# Autodesk Inventor assembly: 566H_plus_Blumotion NL=750 mm Chipboard screws 661.1450.HG 6,3x14,5 L Top row R Top row LD drillings both
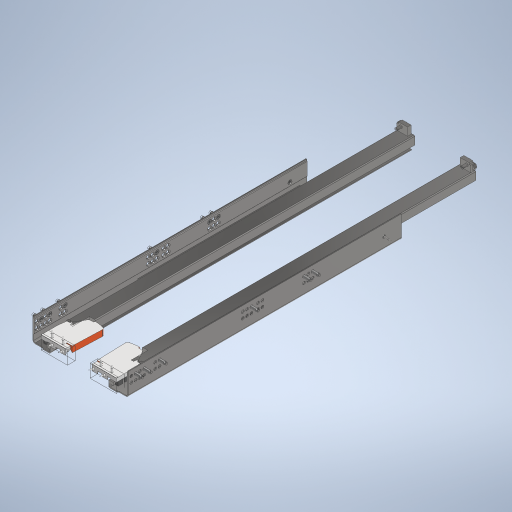
[picture p0: Inventor's stored thumbnail of the model, 512x512]
Saved by Autodesk Inventor 2024 (Build 280153000, 153)
## iProperties
Created: 2019-09-16
Part Number: 566H_plus_Blumotion NL=750 mm Chipboard screws 661.1450.HG 6,3x14,5 L Top row R Top row LD drillings both
Document SubType Name: Assembly
Designer: RokasM
Author: RokasM
## Documents named in this file (296)
- C:\W4INV 2024 Design\LIBRARY\Sliders\Blum TANDEM PLUS BLUMOTION 566 H\566H_iassembly_v1_LD.iam
- C:\W4INV 2024 Design\LIBRARY\Sliders\Blum TANDEM PLUS BLUMOTION 566 H\Blum_TANDEM_PLUS_BLUMOTION_566H.ipt
- C:\W4INV 2024 Design\LIBRARY\Sliders\Blum TANDEM PLUS BLUMOTION 566 H\Lockingdevice.ipt
- C:\W4INV 2024 Design\LIBRARY\Sliders\Blum TANDEM PLUS BLUMOTION 566 H\Locking_device\Locking device L.ipt
- C:\W4INV 2024 Design\LIBRARY\Sliders\Blum TANDEM PLUS BLUMOTION 566 H\Locking_device\Locking device R.ipt
- C:\W4INV 2024 Design\LIBRARY\Sliders\Blum TANDEM PLUS BLUMOTION 566 H\566H\566H7500B01 Chipboard screws top_row L.ipt
- C:\W4INV 2024 Design\LIBRARY\Sliders\Blum TANDEM PLUS BLUMOTION 566 H\566H\566H7500B01 Chipboard screws top_row R.ipt
- C:\W4INV 2020 Design\LIBRARY\Rollers\Blum TANDEM PLUS BLUMOTION 566 H\Lockingdevice.ipt
- 566H_plus_Blumotion NL=450 mm Chipboard screws 4x15 mm L Bottom row R Bottom row LD drillings both.iam
- 566H_plus_Blumotion NL=450 mm Chipboard screws 4x15 mm L Bottom row R Bottom row LD drillings bottom.iam
- 566H_plus_Blumotion NL=450 mm Chipboard screws 4x15 mm L Bottom row R Bottom row LD drillings facade.iam
- 566H_plus_Blumotion NL=450 mm Chipboard screws 4x15 mm L Bottom row R Bottom row LD drillings none.iam
- 566H_plus_Blumotion NL=450 mm Chipboard screws 4x15 mm L Bottom row R Top row LD drillings both.iam
- 566H_plus_Blumotion NL=450 mm Chipboard screws 4x15 mm L Bottom row R Top row LD drillings bottom.iam
- 566H_plus_Blumotion NL=450 mm Chipboard screws 4x15 mm L Bottom row R Top row LD drillings facade.iam
- 566H_plus_Blumotion NL=450 mm Chipboard screws 4x15 mm L Bottom row R Top row LD drillings none.iam
- 566H_plus_Blumotion NL=450 mm Chipboard screws 4x15 mm L Top row R Bottom row LD drillings both.iam
- 566H_plus_Blumotion NL=450 mm Chipboard screws 4x15 mm L Top row R Bottom row LD drillings bottom.iam
- 566H_plus_Blumotion NL=450 mm Chipboard screws 4x15 mm L Top row R Bottom row LD drillings facade.iam
- 566H_plus_Blumotion NL=450 mm Chipboard screws 4x15 mm L Top row R Bottom row LD drillings none.iam
- 566H_plus_Blumotion NL=450 mm Chipboard screws 4x15 mm L Top row R Top row LD drillings both.iam
- 566H_plus_Blumotion NL=450 mm Chipboard screws 4x15 mm L Top row R Top row LD drillings bottom.iam
- 566H_plus_Blumotion NL=450 mm Chipboard screws 4x15 mm L Top row R Top row LD drillings facade.iam
- 566H_plus_Blumotion NL=450 mm Chipboard screws 4x15 mm L Top row R Top row LD drillings none.iam
- 566H_plus_Blumotion NL=450 mm Chipboard screws 661.1450.HG 6,3x14,5 L Bottom row R Bottom row LD drillings both.iam
- 566H_plus_Blumotion NL=450 mm Chipboard screws 661.1450.HG 6,3x14,5 L Bottom row R Bottom row LD drillings bottom.iam
- 566H_plus_Blumotion NL=450 mm Chipboard screws 661.1450.HG 6,3x14,5 L Bottom row R Bottom row LD drillings facade.iam
- 566H_plus_Blumotion NL=450 mm Chipboard screws 661.1450.HG 6,3x14,5 L Bottom row R Bottom row LD drillings none.iam
- 566H_plus_Blumotion NL=450 mm Chipboard screws 661.1450.HG 6,3x14,5 L Bottom row R Top row LD drillings both.iam
- 566H_plus_Blumotion NL=450 mm Chipboard screws 661.1450.HG 6,3x14,5 L Bottom row R Top row LD drillings bottom.iam
- 566H_plus_Blumotion NL=450 mm Chipboard screws 661.1450.HG 6,3x14,5 L Bottom row R Top row LD drillings facade.iam
- 566H_plus_Blumotion NL=450 mm Chipboard screws 661.1450.HG 6,3x14,5 L Bottom row R Top row LD drillings none.iam
- 566H_plus_Blumotion NL=450 mm Chipboard screws 661.1450.HG 6,3x14,5 L Top row R Bottom row LD drillings both.iam
- 566H_plus_Blumotion NL=450 mm Chipboard screws 661.1450.HG 6,3x14,5 L Top row R Bottom row LD drillings bottom.iam
- 566H_plus_Blumotion NL=450 mm Chipboard screws 661.1450.HG 6,3x14,5 L Top row R Bottom row LD drillings facade.iam
- 566H_plus_Blumotion NL=450 mm Chipboard screws 661.1450.HG 6,3x14,5 L Top row R Bottom row LD drillings none.iam
- 566H_plus_Blumotion NL=450 mm Chipboard screws 661.1450.HG 6,3x14,5 L Top row R Top row LD drillings both.iam
- 566H_plus_Blumotion NL=450 mm Chipboard screws 661.1450.HG 6,3x14,5 L Top row R Top row LD drillings bottom.iam
- 566H_plus_Blumotion NL=450 mm Chipboard screws 661.1450.HG 6,3x14,5 L Top row R Top row LD drillings facade.iam
- 566H_plus_Blumotion NL=450 mm Chipboard screws 661.1450.HG 6,3x14,5 L Top row R Top row LD drillings none.iam
- 566H_plus_Blumotion NL=500 mm Chipboard screws 4x15 mm L Bottom row R Bottom row LD drillings both.iam
- 566H_plus_Blumotion NL=500 mm Chipboard screws 4x15 mm L Bottom row R Bottom row LD drillings bottom.iam
- 566H_plus_Blumotion NL=500 mm Chipboard screws 4x15 mm L Bottom row R Bottom row LD drillings facade.iam
- 566H_plus_Blumotion NL=500 mm Chipboard screws 4x15 mm L Bottom row R Bottom row LD drillings none.iam
- 566H_plus_Blumotion NL=500 mm Chipboard screws 4x15 mm L Bottom row R Top row LD drillings both.iam
- 566H_plus_Blumotion NL=500 mm Chipboard screws 4x15 mm L Bottom row R Top row LD drillings bottom.iam
- 566H_plus_Blumotion NL=500 mm Chipboard screws 4x15 mm L Bottom row R Top row LD drillings facade.iam
- 566H_plus_Blumotion NL=500 mm Chipboard screws 4x15 mm L Bottom row R Top row LD drillings none.iam
- 566H_plus_Blumotion NL=500 mm Chipboard screws 4x15 mm L Top row R Bottom row LD drillings both.iam
- 566H_plus_Blumotion NL=500 mm Chipboard screws 4x15 mm L Top row R Bottom row LD drillings bottom.iam
- 566H_plus_Blumotion NL=500 mm Chipboard screws 4x15 mm L Top row R Bottom row LD drillings facade.iam
- 566H_plus_Blumotion NL=500 mm Chipboard screws 4x15 mm L Top row R Bottom row LD drillings none.iam
- 566H_plus_Blumotion NL=500 mm Chipboard screws 4x15 mm L Top row R Top row LD drillings both.iam
- 566H_plus_Blumotion NL=500 mm Chipboard screws 4x15 mm L Top row R Top row LD drillings bottom.iam
- 566H_plus_Blumotion NL=500 mm Chipboard screws 4x15 mm L Top row R Top row LD drillings facade.iam
- 566H_plus_Blumotion NL=500 mm Chipboard screws 4x15 mm L Top row R Top row LD drillings none.iam
- 566H_plus_Blumotion NL=500 mm Chipboard screws 661.1450.HG 6,3x14,5 L Bottom row R Bottom row LD drillings both.iam
- 566H_plus_Blumotion NL=500 mm Chipboard screws 661.1450.HG 6,3x14,5 L Bottom row R Bottom row LD drillings bottom.iam
- 566H_plus_Blumotion NL=500 mm Chipboard screws 661.1450.HG 6,3x14,5 L Bottom row R Bottom row LD drillings facade.iam
- 566H_plus_Blumotion NL=500 mm Chipboard screws 661.1450.HG 6,3x14,5 L Bottom row R Bottom row LD drillings none.iam
- 566H_plus_Blumotion NL=500 mm Chipboard screws 661.1450.HG 6,3x14,5 L Bottom row R Top row LD drillings both.iam
- 566H_plus_Blumotion NL=500 mm Chipboard screws 661.1450.HG 6,3x14,5 L Bottom row R Top row LD drillings bottom.iam
- 566H_plus_Blumotion NL=500 mm Chipboard screws 661.1450.HG 6,3x14,5 L Bottom row R Top row LD drillings facade.iam
- 566H_plus_Blumotion NL=500 mm Chipboard screws 661.1450.HG 6,3x14,5 L Bottom row R Top row LD drillings none.iam
- 566H_plus_Blumotion NL=500 mm Chipboard screws 661.1450.HG 6,3x14,5 L Top row R Bottom row LD drillings both.iam
- 566H_plus_Blumotion NL=500 mm Chipboard screws 661.1450.HG 6,3x14,5 L Top row R Bottom row LD drillings bottom.iam
- 566H_plus_Blumotion NL=500 mm Chipboard screws 661.1450.HG 6,3x14,5 L Top row R Bottom row LD drillings facade.iam
- 566H_plus_Blumotion NL=500 mm Chipboard screws 661.1450.HG 6,3x14,5 L Top row R Bottom row LD drillings none.iam
- 566H_plus_Blumotion NL=500 mm Chipboard screws 661.1450.HG 6,3x14,5 L Top row R Top row LD drillings both.iam
- 566H_plus_Blumotion NL=500 mm Chipboard screws 661.1450.HG 6,3x14,5 L Top row R Top row LD drillings bottom.iam
- 566H_plus_Blumotion NL=500 mm Chipboard screws 661.1450.HG 6,3x14,5 L Top row R Top row LD drillings facade.iam
- 566H_plus_Blumotion NL=500 mm Chipboard screws 661.1450.HG 6,3x14,5 L Top row R Top row LD drillings none.iam
- 566H_plus_Blumotion NL=520 mm Chipboard screws 4x15 mm L Bottom row R Bottom row LD drillings both.iam
- 566H_plus_Blumotion NL=520 mm Chipboard screws 4x15 mm L Bottom row R Bottom row LD drillings bottom.iam
- 566H_plus_Blumotion NL=520 mm Chipboard screws 4x15 mm L Bottom row R Bottom row LD drillings facade.iam
- 566H_plus_Blumotion NL=520 mm Chipboard screws 4x15 mm L Bottom row R Bottom row LD drillings none.iam
- 566H_plus_Blumotion NL=520 mm Chipboard screws 4x15 mm L Bottom row R Top row LD drillings both.iam
- 566H_plus_Blumotion NL=520 mm Chipboard screws 4x15 mm L Bottom row R Top row LD drillings bottom.iam
- 566H_plus_Blumotion NL=520 mm Chipboard screws 4x15 mm L Bottom row R Top row LD drillings facade.iam
- 566H_plus_Blumotion NL=520 mm Chipboard screws 4x15 mm L Bottom row R Top row LD drillings none.iam
- 566H_plus_Blumotion NL=520 mm Chipboard screws 4x15 mm L Top row R Bottom row LD drillings both.iam
- 566H_plus_Blumotion NL=520 mm Chipboard screws 4x15 mm L Top row R Bottom row LD drillings bottom.iam
- 566H_plus_Blumotion NL=520 mm Chipboard screws 4x15 mm L Top row R Bottom row LD drillings facade.iam
- 566H_plus_Blumotion NL=520 mm Chipboard screws 4x15 mm L Top row R Bottom row LD drillings none.iam
- 566H_plus_Blumotion NL=520 mm Chipboard screws 4x15 mm L Top row R Top row LD drillings both.iam
- 566H_plus_Blumotion NL=520 mm Chipboard screws 4x15 mm L Top row R Top row LD drillings bottom.iam
- 566H_plus_Blumotion NL=520 mm Chipboard screws 4x15 mm L Top row R Top row LD drillings facade.iam
- 566H_plus_Blumotion NL=520 mm Chipboard screws 4x15 mm L Top row R Top row LD drillings none.iam
- 566H_plus_Blumotion NL=520 mm Chipboard screws 661.1450.HG 6,3x14,5 L Bottom row R Bottom row LD drillings both.iam
- 566H_plus_Blumotion NL=520 mm Chipboard screws 661.1450.HG 6,3x14,5 L Bottom row R Bottom row LD drillings bottom.iam
- 566H_plus_Blumotion NL=520 mm Chipboard screws 661.1450.HG 6,3x14,5 L Bottom row R Bottom row LD drillings facade.iam
- 566H_plus_Blumotion NL=520 mm Chipboard screws 661.1450.HG 6,3x14,5 L Bottom row R Bottom row LD drillings none.iam
- 566H_plus_Blumotion NL=520 mm Chipboard screws 661.1450.HG 6,3x14,5 L Bottom row R Top row LD drillings both.iam
- 566H_plus_Blumotion NL=520 mm Chipboard screws 661.1450.HG 6,3x14,5 L Bottom row R Top row LD drillings bottom.iam
- 566H_plus_Blumotion NL=520 mm Chipboard screws 661.1450.HG 6,3x14,5 L Bottom row R Top row LD drillings facade.iam
- 566H_plus_Blumotion NL=520 mm Chipboard screws 661.1450.HG 6,3x14,5 L Bottom row R Top row LD drillings none.iam
- 566H_plus_Blumotion NL=520 mm Chipboard screws 661.1450.HG 6,3x14,5 L Top row R Bottom row LD drillings both.iam
- 566H_plus_Blumotion NL=520 mm Chipboard screws 661.1450.HG 6,3x14,5 L Top row R Bottom row LD drillings bottom.iam
- 566H_plus_Blumotion NL=520 mm Chipboard screws 661.1450.HG 6,3x14,5 L Top row R Bottom row LD drillings facade.iam
- 566H_plus_Blumotion NL=520 mm Chipboard screws 661.1450.HG 6,3x14,5 L Top row R Bottom row LD drillings none.iam
- 566H_plus_Blumotion NL=520 mm Chipboard screws 661.1450.HG 6,3x14,5 L Top row R Top row LD drillings both.iam
- 566H_plus_Blumotion NL=520 mm Chipboard screws 661.1450.HG 6,3x14,5 L Top row R Top row LD drillings bottom.iam
- 566H_plus_Blumotion NL=520 mm Chipboard screws 661.1450.HG 6,3x14,5 L Top row R Top row LD drillings facade.iam
- 566H_plus_Blumotion NL=520 mm Chipboard screws 661.1450.HG 6,3x14,5 L Top row R Top row LD drillings none.iam
- 566H_plus_Blumotion NL=550 mm Chipboard screws 4x15 mm L Bottom row R Bottom row LD drillings both.iam
- 566H_plus_Blumotion NL=550 mm Chipboard screws 4x15 mm L Bottom row R Bottom row LD drillings bottom.iam
- 566H_plus_Blumotion NL=550 mm Chipboard screws 4x15 mm L Bottom row R Bottom row LD drillings facade.iam
- 566H_plus_Blumotion NL=550 mm Chipboard screws 4x15 mm L Bottom row R Bottom row LD drillings none.iam
- 566H_plus_Blumotion NL=550 mm Chipboard screws 4x15 mm L Bottom row R Top row LD drillings both.iam
- 566H_plus_Blumotion NL=550 mm Chipboard screws 4x15 mm L Bottom row R Top row LD drillings bottom.iam
- 566H_plus_Blumotion NL=550 mm Chipboard screws 4x15 mm L Bottom row R Top row LD drillings facade.iam
- 566H_plus_Blumotion NL=550 mm Chipboard screws 4x15 mm L Bottom row R Top row LD drillings none.iam
- 566H_plus_Blumotion NL=550 mm Chipboard screws 4x15 mm L Top row R Bottom row LD drillings both.iam
- 566H_plus_Blumotion NL=550 mm Chipboard screws 4x15 mm L Top row R Bottom row LD drillings bottom.iam
- 566H_plus_Blumotion NL=550 mm Chipboard screws 4x15 mm L Top row R Bottom row LD drillings facade.iam
- 566H_plus_Blumotion NL=550 mm Chipboard screws 4x15 mm L Top row R Bottom row LD drillings none.iam
- 566H_plus_Blumotion NL=550 mm Chipboard screws 4x15 mm L Top row R Top row LD drillings both.iam
- 566H_plus_Blumotion NL=550 mm Chipboard screws 4x15 mm L Top row R Top row LD drillings bottom.iam
- 566H_plus_Blumotion NL=550 mm Chipboard screws 4x15 mm L Top row R Top row LD drillings facade.iam
- 566H_plus_Blumotion NL=550 mm Chipboard screws 4x15 mm L Top row R Top row LD drillings none.iam
- 566H_plus_Blumotion NL=550 mm Chipboard screws 661.1450.HG 6,3x14,5 L Bottom row R Bottom row LD drillings both.iam
- 566H_plus_Blumotion NL=550 mm Chipboard screws 661.1450.HG 6,3x14,5 L Bottom row R Bottom row LD drillings bottom.iam
- 566H_plus_Blumotion NL=550 mm Chipboard screws 661.1450.HG 6,3x14,5 L Bottom row R Bottom row LD drillings facade.iam
- 566H_plus_Blumotion NL=550 mm Chipboard screws 661.1450.HG 6,3x14,5 L Bottom row R Bottom row LD drillings none.iam
- 566H_plus_Blumotion NL=550 mm Chipboard screws 661.1450.HG 6,3x14,5 L Bottom row R Top row LD drillings both.iam
- 566H_plus_Blumotion NL=550 mm Chipboard screws 661.1450.HG 6,3x14,5 L Bottom row R Top row LD drillings bottom.iam
- 566H_plus_Blumotion NL=550 mm Chipboard screws 661.1450.HG 6,3x14,5 L Bottom row R Top row LD drillings facade.iam
- 566H_plus_Blumotion NL=550 mm Chipboard screws 661.1450.HG 6,3x14,5 L Bottom row R Top row LD drillings none.iam
- 566H_plus_Blumotion NL=550 mm Chipboard screws 661.1450.HG 6,3x14,5 L Top row R Bottom row LD drillings both.iam
- 566H_plus_Blumotion NL=550 mm Chipboard screws 661.1450.HG 6,3x14,5 L Top row R Bottom row LD drillings bottom.iam
- 566H_plus_Blumotion NL=550 mm Chipboard screws 661.1450.HG 6,3x14,5 L Top row R Bottom row LD drillings facade.iam
- 566H_plus_Blumotion NL=550 mm Chipboard screws 661.1450.HG 6,3x14,5 L Top row R Bottom row LD drillings none.iam
- 566H_plus_Blumotion NL=550 mm Chipboard screws 661.1450.HG 6,3x14,5 L Top row R Top row LD drillings both.iam
- 566H_plus_Blumotion NL=550 mm Chipboard screws 661.1450.HG 6,3x14,5 L Top row R Top row LD drillings bottom.iam
- 566H_plus_Blumotion NL=550 mm Chipboard screws 661.1450.HG 6,3x14,5 L Top row R Top row LD drillings facade.iam
- 566H_plus_Blumotion NL=550 mm Chipboard screws 661.1450.HG 6,3x14,5 L Top row R Top row LD drillings none.iam
- 566H_plus_Blumotion NL=580 mm Chipboard screws 4x15 mm L Bottom row R Bottom row LD drillings both.iam
- 566H_plus_Blumotion NL=580 mm Chipboard screws 4x15 mm L Bottom row R Bottom row LD drillings bottom.iam
- 566H_plus_Blumotion NL=580 mm Chipboard screws 4x15 mm L Bottom row R Bottom row LD drillings facade.iam
- 566H_plus_Blumotion NL=580 mm Chipboard screws 4x15 mm L Bottom row R Bottom row LD drillings none.iam
- 566H_plus_Blumotion NL=580 mm Chipboard screws 4x15 mm L Bottom row R Top row LD drillings both.iam
- 566H_plus_Blumotion NL=580 mm Chipboard screws 4x15 mm L Bottom row R Top row LD drillings bottom.iam
- 566H_plus_Blumotion NL=580 mm Chipboard screws 4x15 mm L Bottom row R Top row LD drillings facade.iam
- 566H_plus_Blumotion NL=580 mm Chipboard screws 4x15 mm L Bottom row R Top row LD drillings none.iam
- 566H_plus_Blumotion NL=580 mm Chipboard screws 4x15 mm L Top row R Bottom row LD drillings both.iam
- 566H_plus_Blumotion NL=580 mm Chipboard screws 4x15 mm L Top row R Bottom row LD drillings bottom.iam
- 566H_plus_Blumotion NL=580 mm Chipboard screws 4x15 mm L Top row R Bottom row LD drillings facade.iam
- 566H_plus_Blumotion NL=580 mm Chipboard screws 4x15 mm L Top row R Bottom row LD drillings none.iam
- 566H_plus_Blumotion NL=580 mm Chipboard screws 4x15 mm L Top row R Top row LD drillings both.iam
- 566H_plus_Blumotion NL=580 mm Chipboard screws 4x15 mm L Top row R Top row LD drillings bottom.iam
- 566H_plus_Blumotion NL=580 mm Chipboard screws 4x15 mm L Top row R Top row LD drillings facade.iam
- 566H_plus_Blumotion NL=580 mm Chipboard screws 4x15 mm L Top row R Top row LD drillings none.iam
- 566H_plus_Blumotion NL=580 mm Chipboard screws 661.1450.HG 6,3x14,5 L Bottom row R Bottom row LD drillings both.iam
- 566H_plus_Blumotion NL=580 mm Chipboard screws 661.1450.HG 6,3x14,5 L Bottom row R Bottom row LD drillings bottom.iam
- 566H_plus_Blumotion NL=580 mm Chipboard screws 661.1450.HG 6,3x14,5 L Bottom row R Bottom row LD drillings facade.iam
- 566H_plus_Blumotion NL=580 mm Chipboard screws 661.1450.HG 6,3x14,5 L Bottom row R Bottom row LD drillings none.iam
- 566H_plus_Blumotion NL=580 mm Chipboard screws 661.1450.HG 6,3x14,5 L Bottom row R Top row LD drillings both.iam
- 566H_plus_Blumotion NL=580 mm Chipboard screws 661.1450.HG 6,3x14,5 L Bottom row R Top row LD drillings bottom.iam
- 566H_plus_Blumotion NL=580 mm Chipboard screws 661.1450.HG 6,3x14,5 L Bottom row R Top row LD drillings facade.iam
- 566H_plus_Blumotion NL=580 mm Chipboard screws 661.1450.HG 6,3x14,5 L Bottom row R Top row LD drillings none.iam
- 566H_plus_Blumotion NL=580 mm Chipboard screws 661.1450.HG 6,3x14,5 L Top row R Bottom row LD drillings both.iam
- 566H_plus_Blumotion NL=580 mm Chipboard screws 661.1450.HG 6,3x14,5 L Top row R Bottom row LD drillings bottom.iam
- 566H_plus_Blumotion NL=580 mm Chipboard screws 661.1450.HG 6,3x14,5 L Top row R Bottom row LD drillings facade.iam
- 566H_plus_Blumotion NL=580 mm Chipboard screws 661.1450.HG 6,3x14,5 L Top row R Bottom row LD drillings none.iam
- 566H_plus_Blumotion NL=580 mm Chipboard screws 661.1450.HG 6,3x14,5 L Top row R Top row LD drillings both.iam
- 566H_plus_Blumotion NL=580 mm Chipboard screws 661.1450.HG 6,3x14,5 L Top row R Top row LD drillings bottom.iam
- 566H_plus_Blumotion NL=580 mm Chipboard screws 661.1450.HG 6,3x14,5 L Top row R Top row LD drillings facade.iam
- 566H_plus_Blumotion NL=580 mm Chipboard screws 661.1450.HG 6,3x14,5 L Top row R Top row LD drillings none.iam
- 566H_plus_Blumotion NL=600 mm Chipboard screws 4x15 mm L Bottom row R Bottom row LD drillings both.iam
- 566H_plus_Blumotion NL=600 mm Chipboard screws 4x15 mm L Bottom row R Bottom row LD drillings bottom.iam
- 566H_plus_Blumotion NL=600 mm Chipboard screws 4x15 mm L Bottom row R Bottom row LD drillings facade.iam
- 566H_plus_Blumotion NL=600 mm Chipboard screws 4x15 mm L Bottom row R Bottom row LD drillings none.iam
- 566H_plus_Blumotion NL=600 mm Chipboard screws 4x15 mm L Bottom row R Top row LD drillings both.iam
- 566H_plus_Blumotion NL=600 mm Chipboard screws 4x15 mm L Bottom row R Top row LD drillings bottom.iam
- 566H_plus_Blumotion NL=600 mm Chipboard screws 4x15 mm L Bottom row R Top row LD drillings facade.iam
- 566H_plus_Blumotion NL=600 mm Chipboard screws 4x15 mm L Bottom row R Top row LD drillings none.iam
- 566H_plus_Blumotion NL=600 mm Chipboard screws 4x15 mm L Top row R Bottom row LD drillings both.iam
- 566H_plus_Blumotion NL=600 mm Chipboard screws 4x15 mm L Top row R Bottom row LD drillings bottom.iam
- 566H_plus_Blumotion NL=600 mm Chipboard screws 4x15 mm L Top row R Bottom row LD drillings facade.iam
- 566H_plus_Blumotion NL=600 mm Chipboard screws 4x15 mm L Top row R Bottom row LD drillings none.iam
- 566H_plus_Blumotion NL=600 mm Chipboard screws 4x15 mm L Top row R Top row LD drillings both.iam
- 566H_plus_Blumotion NL=600 mm Chipboard screws 4x15 mm L Top row R Top row LD drillings bottom.iam
- 566H_plus_Blumotion NL=600 mm Chipboard screws 4x15 mm L Top row R Top row LD drillings facade.iam
- 566H_plus_Blumotion NL=600 mm Chipboard screws 4x15 mm L Top row R Top row LD drillings none.iam
- 566H_plus_Blumotion NL=600 mm Chipboard screws 661.1450.HG 6,3x14,5 L Bottom row R Bottom row LD drillings both.iam
- 566H_plus_Blumotion NL=600 mm Chipboard screws 661.1450.HG 6,3x14,5 L Bottom row R Bottom row LD drillings bottom.iam
- 566H_plus_Blumotion NL=600 mm Chipboard screws 661.1450.HG 6,3x14,5 L Bottom row R Bottom row LD drillings facade.iam
- 566H_plus_Blumotion NL=600 mm Chipboard screws 661.1450.HG 6,3x14,5 L Bottom row R Bottom row LD drillings none.iam
- 566H_plus_Blumotion NL=600 mm Chipboard screws 661.1450.HG 6,3x14,5 L Bottom row R Top row LD drillings both.iam
- 566H_plus_Blumotion NL=600 mm Chipboard screws 661.1450.HG 6,3x14,5 L Bottom row R Top row LD drillings bottom.iam
- 566H_plus_Blumotion NL=600 mm Chipboard screws 661.1450.HG 6,3x14,5 L Bottom row R Top row LD drillings facade.iam
- 566H_plus_Blumotion NL=600 mm Chipboard screws 661.1450.HG 6,3x14,5 L Bottom row R Top row LD drillings none.iam
- 566H_plus_Blumotion NL=600 mm Chipboard screws 661.1450.HG 6,3x14,5 L Top row R Bottom row LD drillings both.iam
- 566H_plus_Blumotion NL=600 mm Chipboard screws 661.1450.HG 6,3x14,5 L Top row R Bottom row LD drillings bottom.iam
- 566H_plus_Blumotion NL=600 mm Chipboard screws 661.1450.HG 6,3x14,5 L Top row R Bottom row LD drillings facade.iam
- 566H_plus_Blumotion NL=600 mm Chipboard screws 661.1450.HG 6,3x14,5 L Top row R Bottom row LD drillings none.iam
- 566H_plus_Blumotion NL=600 mm Chipboard screws 661.1450.HG 6,3x14,5 L Top row R Top row LD drillings both.iam
- 566H_plus_Blumotion NL=600 mm Chipboard screws 661.1450.HG 6,3x14,5 L Top row R Top row LD drillings bottom.iam
- 566H_plus_Blumotion NL=600 mm Chipboard screws 661.1450.HG 6,3x14,5 L Top row R Top row LD drillings facade.iam
- 566H_plus_Blumotion NL=600 mm Chipboard screws 661.1450.HG 6,3x14,5 L Top row R Top row LD drillings none.iam
- 566H_plus_Blumotion NL=650 mm Chipboard screws 4x15 mm L Bottom row R Bottom row LD drillings both.iam
- 566H_plus_Blumotion NL=650 mm Chipboard screws 4x15 mm L Bottom row R Bottom row LD drillings bottom.iam
- 566H_plus_Blumotion NL=650 mm Chipboard screws 4x15 mm L Bottom row R Bottom row LD drillings facade.iam
- 566H_plus_Blumotion NL=650 mm Chipboard screws 4x15 mm L Bottom row R Bottom row LD drillings none.iam
- 566H_plus_Blumotion NL=650 mm Chipboard screws 4x15 mm L Bottom row R Top row LD drillings both.iam
- 566H_plus_Blumotion NL=650 mm Chipboard screws 4x15 mm L Bottom row R Top row LD drillings bottom.iam
- 566H_plus_Blumotion NL=650 mm Chipboard screws 4x15 mm L Bottom row R Top row LD drillings facade.iam
- 566H_plus_Blumotion NL=650 mm Chipboard screws 4x15 mm L Bottom row R Top row LD drillings none.iam
- 566H_plus_Blumotion NL=650 mm Chipboard screws 4x15 mm L Top row R Bottom row LD drillings both.iam
- 566H_plus_Blumotion NL=650 mm Chipboard screws 4x15 mm L Top row R Bottom row LD drillings bottom.iam
- 566H_plus_Blumotion NL=650 mm Chipboard screws 4x15 mm L Top row R Bottom row LD drillings facade.iam
- 566H_plus_Blumotion NL=650 mm Chipboard screws 4x15 mm L Top row R Bottom row LD drillings none.iam
- 566H_plus_Blumotion NL=650 mm Chipboard screws 4x15 mm L Top row R Top row LD drillings both.iam
- 566H_plus_Blumotion NL=650 mm Chipboard screws 4x15 mm L Top row R Top row LD drillings bottom.iam
- 566H_plus_Blumotion NL=650 mm Chipboard screws 4x15 mm L Top row R Top row LD drillings facade.iam
- 566H_plus_Blumotion NL=650 mm Chipboard screws 4x15 mm L Top row R Top row LD drillings none.iam
- 566H_plus_Blumotion NL=650 mm Chipboard screws 661.1450.HG 6,3x14,5 L Bottom row R Bottom row LD drillings both.iam
- 566H_plus_Blumotion NL=650 mm Chipboard screws 661.1450.HG 6,3x14,5 L Bottom row R Bottom row LD drillings bottom.iam
- 566H_plus_Blumotion NL=650 mm Chipboard screws 661.1450.HG 6,3x14,5 L Bottom row R Bottom row LD drillings facade.iam
- 566H_plus_Blumotion NL=650 mm Chipboard screws 661.1450.HG 6,3x14,5 L Bottom row R Bottom row LD drillings none.iam
- 566H_plus_Blumotion NL=650 mm Chipboard screws 661.1450.HG 6,3x14,5 L Bottom row R Top row LD drillings both.iam
- 566H_plus_Blumotion NL=650 mm Chipboard screws 661.1450.HG 6,3x14,5 L Bottom row R Top row LD drillings bottom.iam
- 566H_plus_Blumotion NL=650 mm Chipboard screws 661.1450.HG 6,3x14,5 L Bottom row R Top row LD drillings facade.iam
- 566H_plus_Blumotion NL=650 mm Chipboard screws 661.1450.HG 6,3x14,5 L Bottom row R Top row LD drillings none.iam
- 566H_plus_Blumotion NL=650 mm Chipboard screws 661.1450.HG 6,3x14,5 L Top row R Bottom row LD drillings both.iam
- 566H_plus_Blumotion NL=650 mm Chipboard screws 661.1450.HG 6,3x14,5 L Top row R Bottom row LD drillings bottom.iam
- 566H_plus_Blumotion NL=650 mm Chipboard screws 661.1450.HG 6,3x14,5 L Top row R Bottom row LD drillings facade.iam
- 566H_plus_Blumotion NL=650 mm Chipboard screws 661.1450.HG 6,3x14,5 L Top row R Bottom row LD drillings none.iam
- 566H_plus_Blumotion NL=650 mm Chipboard screws 661.1450.HG 6,3x14,5 L Top row R Top row LD drillings both.iam
- 566H_plus_Blumotion NL=650 mm Chipboard screws 661.1450.HG 6,3x14,5 L Top row R Top row LD drillings bottom.iam
- 566H_plus_Blumotion NL=650 mm Chipboard screws 661.1450.HG 6,3x14,5 L Top row R Top row LD drillings facade.iam
- 566H_plus_Blumotion NL=650 mm Chipboard screws 661.1450.HG 6,3x14,5 L Top row R Top row LD drillings none.iam
- 566H_plus_Blumotion NL=700 mm Chipboard screws 4x15 mm L Bottom row R Bottom row LD drillings both.iam
- 566H_plus_Blumotion NL=700 mm Chipboard screws 4x15 mm L Bottom row R Bottom row LD drillings bottom.iam
- 566H_plus_Blumotion NL=700 mm Chipboard screws 4x15 mm L Bottom row R Bottom row LD drillings facade.iam
- 566H_plus_Blumotion NL=700 mm Chipboard screws 4x15 mm L Bottom row R Bottom row LD drillings none.iam
- 566H_plus_Blumotion NL=700 mm Chipboard screws 4x15 mm L Bottom row R Top row LD drillings both.iam
- 566H_plus_Blumotion NL=700 mm Chipboard screws 4x15 mm L Bottom row R Top row LD drillings bottom.iam
- 566H_plus_Blumotion NL=700 mm Chipboard screws 4x15 mm L Bottom row R Top row LD drillings facade.iam
- 566H_plus_Blumotion NL=700 mm Chipboard screws 4x15 mm L Bottom row R Top row LD drillings none.iam
- 566H_plus_Blumotion NL=700 mm Chipboard screws 4x15 mm L Top row R Bottom row LD drillings both.iam
- 566H_plus_Blumotion NL=700 mm Chipboard screws 4x15 mm L Top row R Bottom row LD drillings bottom.iam
- 566H_plus_Blumotion NL=700 mm Chipboard screws 4x15 mm L Top row R Bottom row LD drillings facade.iam
- 566H_plus_Blumotion NL=700 mm Chipboard screws 4x15 mm L Top row R Bottom row LD drillings none.iam
- 566H_plus_Blumotion NL=700 mm Chipboard screws 4x15 mm L Top row R Top row LD drillings both.iam
- 566H_plus_Blumotion NL=700 mm Chipboard screws 4x15 mm L Top row R Top row LD drillings bottom.iam
- 566H_plus_Blumotion NL=700 mm Chipboard screws 4x15 mm L Top row R Top row LD drillings facade.iam
- 566H_plus_Blumotion NL=700 mm Chipboard screws 4x15 mm L Top row R Top row LD drillings none.iam
- 566H_plus_Blumotion NL=700 mm Chipboard screws 661.1450.HG 6,3x14,5 L Bottom row R Bottom row LD drillings both.iam
- 566H_plus_Blumotion NL=700 mm Chipboard screws 661.1450.HG 6,3x14,5 L Bottom row R Bottom row LD drillings bottom.iam
- 566H_plus_Blumotion NL=700 mm Chipboard screws 661.1450.HG 6,3x14,5 L Bottom row R Bottom row LD drillings facade.iam
- 566H_plus_Blumotion NL=700 mm Chipboard screws 661.1450.HG 6,3x14,5 L Bottom row R Bottom row LD drillings none.iam
- 566H_plus_Blumotion NL=700 mm Chipboard screws 661.1450.HG 6,3x14,5 L Bottom row R Top row LD drillings both.iam
- 566H_plus_Blumotion NL=700 mm Chipboard screws 661.1450.HG 6,3x14,5 L Bottom row R Top row LD drillings bottom.iam
- 566H_plus_Blumotion NL=700 mm Chipboard screws 661.1450.HG 6,3x14,5 L Bottom row R Top row LD drillings facade.iam
- 566H_plus_Blumotion NL=700 mm Chipboard screws 661.1450.HG 6,3x14,5 L Bottom row R Top row LD drillings none.iam
- 566H_plus_Blumotion NL=700 mm Chipboard screws 661.1450.HG 6,3x14,5 L Top row R Bottom row LD drillings both.iam
- 566H_plus_Blumotion NL=700 mm Chipboard screws 661.1450.HG 6,3x14,5 L Top row R Bottom row LD drillings bottom.iam
- 566H_plus_Blumotion NL=700 mm Chipboard screws 661.1450.HG 6,3x14,5 L Top row R Bottom row LD drillings facade.iam
- 566H_plus_Blumotion NL=700 mm Chipboard screws 661.1450.HG 6,3x14,5 L Top row R Bottom row LD drillings none.iam
- 566H_plus_Blumotion NL=700 mm Chipboard screws 661.1450.HG 6,3x14,5 L Top row R Top row LD drillings both.iam
- 566H_plus_Blumotion NL=700 mm Chipboard screws 661.1450.HG 6,3x14,5 L Top row R Top row LD drillings bottom.iam
- 566H_plus_Blumotion NL=700 mm Chipboard screws 661.1450.HG 6,3x14,5 L Top row R Top row LD drillings facade.iam
- 566H_plus_Blumotion NL=700 mm Chipboard screws 661.1450.HG 6,3x14,5 L Top row R Top row LD drillings none.iam
- 566H_plus_Blumotion NL=750 mm Chipboard screws 4x15 mm L Bottom row R Bottom row LD drillings both.iam
- 566H_plus_Blumotion NL=750 mm Chipboard screws 4x15 mm L Bottom row R Bottom row LD drillings bottom.iam
- 566H_plus_Blumotion NL=750 mm Chipboard screws 4x15 mm L Bottom row R Bottom row LD drillings facade.iam
- 566H_plus_Blumotion NL=750 mm Chipboard screws 4x15 mm L Bottom row R Bottom row LD drillings none.iam
- 566H_plus_Blumotion NL=750 mm Chipboard screws 4x15 mm L Bottom row R Top row LD drillings both.iam
- 566H_plus_Blumotion NL=750 mm Chipboard screws 4x15 mm L Bottom row R Top row LD drillings bottom.iam
- 566H_plus_Blumotion NL=750 mm Chipboard screws 4x15 mm L Bottom row R Top row LD drillings facade.iam
- 566H_plus_Blumotion NL=750 mm Chipboard screws 4x15 mm L Bottom row R Top row LD drillings none.iam
- 566H_plus_Blumotion NL=750 mm Chipboard screws 4x15 mm L Top row R Bottom row LD drillings both.iam
- 566H_plus_Blumotion NL=750 mm Chipboard screws 4x15 mm L Top row R Bottom row LD drillings bottom.iam
- 566H_plus_Blumotion NL=750 mm Chipboard screws 4x15 mm L Top row R Bottom row LD drillings facade.iam
- 566H_plus_Blumotion NL=750 mm Chipboard screws 4x15 mm L Top row R Bottom row LD drillings none.iam
- 566H_plus_Blumotion NL=750 mm Chipboard screws 4x15 mm L Top row R Top row LD drillings both.iam
- 566H_plus_Blumotion NL=750 mm Chipboard screws 4x15 mm L Top row R Top row LD drillings bottom.iam
- 566H_plus_Blumotion NL=750 mm Chipboard screws 4x15 mm L Top row R Top row LD drillings facade.iam
- 566H_plus_Blumotion NL=750 mm Chipboard screws 4x15 mm L Top row R Top row LD drillings none.iam
- 566H_plus_Blumotion NL=750 mm Chipboard screws 661.1450.HG 6,3x14,5 L Bottom row R Bottom row LD drillings both.iam
- 566H_plus_Blumotion NL=750 mm Chipboard screws 661.1450.HG 6,3x14,5 L Bottom row R Bottom row LD drillings bottom.iam
- 566H_plus_Blumotion NL=750 mm Chipboard screws 661.1450.HG 6,3x14,5 L Bottom row R Bottom row LD drillings facade.iam
- 566H_plus_Blumotion NL=750 mm Chipboard screws 661.1450.HG 6,3x14,5 L Bottom row R Bottom row LD drillings none.iam
- 566H_plus_Blumotion NL=750 mm Chipboard screws 661.1450.HG 6,3x14,5 L Bottom row R Top row LD drillings both.iam
- 566H_plus_Blumotion NL=750 mm Chipboard screws 661.1450.HG 6,3x14,5 L Bottom row R Top row LD drillings bottom.iam
- 566H_plus_Blumotion NL=750 mm Chipboard screws 661.1450.HG 6,3x14,5 L Bottom row R Top row LD drillings facade.iam
- 566H_plus_Blumotion NL=750 mm Chipboard screws 661.1450.HG 6,3x14,5 L Bottom row R Top row LD drillings none.iam
- 566H_plus_Blumotion NL=750 mm Chipboard screws 661.1450.HG 6,3x14,5 L Top row R Bottom row LD drillings both.iam
- 566H_plus_Blumotion NL=750 mm Chipboard screws 661.1450.HG 6,3x14,5 L Top row R Bottom row LD drillings bottom.iam
- 566H_plus_Blumotion NL=750 mm Chipboard screws 661.1450.HG 6,3x14,5 L Top row R Bottom row LD drillings facade.iam
- 566H_plus_Blumotion NL=750 mm Chipboard screws 661.1450.HG 6,3x14,5 L Top row R Bottom row LD drillings none.iam
- 566H_plus_Blumotion NL=750 mm Chipboard screws 661.1450.HG 6,3x14,5 L Top row R Top row LD drillings both.iam
- 566H_plus_Blumotion NL=750 mm Chipboard screws 661.1450.HG 6,3x14,5 L Top row R Top row LD drillings bottom.iam
- 566H_plus_Blumotion NL=750 mm Chipboard screws 661.1450.HG 6,3x14,5 L Top row R Top row LD drillings facade.iam
- 566H_plus_Blumotion NL=750 mm Chipboard screws 661.1450.HG 6,3x14,5 L Top row R Top row LD drillings none.iam
## Components (4 placed, 4 different names)
1. 566H7500B01 Chipboard screws top_row L:1 — Flush:1, Flush:2, Flush:3, Flush:7
2. 566H7500B01 Chipboard screws top_row R:2 — Flush:1, Flush:2, Flush:4, Flush:8
3. Locking device L:1 — Flush:3, Flush:5, Flush:6, Flush:7
4. Locking device R:2 — Flush:4, Flush:5, Flush:6, Flush:8
## Relationships (8: Flush 8)
- Flush:1: 566H7500B01 Chipboard screws top_row L:1 ↔ 566H7500B01 Chipboard screws top_row R:2
- Flush:2: 566H7500B01 Chipboard screws top_row L:1 ↔ 566H7500B01 Chipboard screws top_row R:2
- Flush:3: 566H7500B01 Chipboard screws top_row L:1 ↔ Locking device L:1
- Flush:4: 566H7500B01 Chipboard screws top_row R:2 ↔ Locking device R:2
- Flush:5: Locking device L:1 ↔ Locking device R:2
- Flush:6: Locking device L:1 ↔ Locking device R:2
- Flush:7 (-2 mm): 566H7500B01 Chipboard screws top_row L:1 ↔ Locking device L:1
- Flush:8: 566H7500B01 Chipboard screws top_row R:2 ↔ Locking device R:2
